# Autodesk Inventor assembly: SMALLER
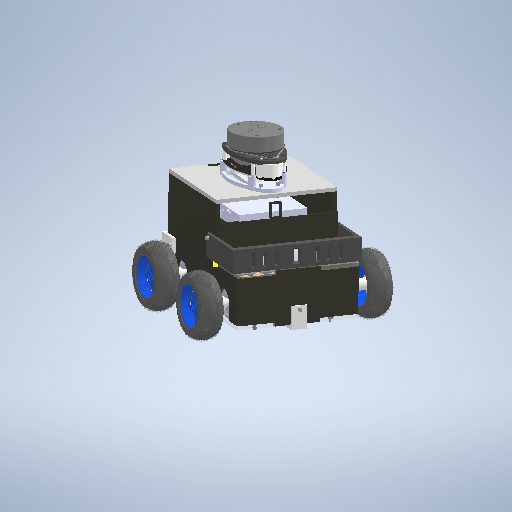
[picture p0: Inventor's stored thumbnail of the model, 512x512]
Saved by Autodesk Inventor 2025.3 (Build 293356030, 356C)
## iProperties
Created: 2026-06-30
Part Number: SMALLER
Document SubType Name: Assembly
Designer: user
Author: user
## Documents named in this file (14)
- C:\Users\user\Downloads\final_design\amy_robot_design.iam
- C:\Users\user\Downloads\final_design\motor_wheel\wheel_base.iam
- C:\Users\user\Downloads\final_design\chassis_boards\back.ipt
- C:\Users\user\Downloads\final_design\chassis_boards\Fastener.ipt
- C:\Users\user\Downloads\final_design\chassis_boards\side.ipt
- C:\Users\user\Downloads\final_design\chassis_boards\hood.ipt
- C:\Users\user\Downloads\final_design\chassis_boards\top.ipt
- C:\Users\user\Downloads\final_design\chassis_boards\front.ipt
- C:\Users\user\Downloads\final_design\chassis_boards\cover.ipt
- C:\Users\user\Downloads\final_design\chassis_boards\holder.ipt
- C:\Docs\shcool\dojo\CAD_stuff\Imports\assembled_lidar.iam
- C:\Docs\shcool\dojo\CAD_stuff\Design_3 - Copy\pi_internals\Complete_model.iam
- C:\Users\user\OneDrive\Documents\Inventor\Content Center Files\R2025\en-US\ISO 7040\DIEN EN ISO 7040 - M3.ipt
- C:\Users\user\OneDrive\Documents\Inventor\Content Center Files\R2025\en-US\ISO 4762(2)\ISO 4762 - M3 x 16ISO.ipt
## Components (48 placed, 13 different names)
1. wheel_base:1 [sub-assembly] — Mate:15, Mate:16, Mate:17, Mate:18, Mate:19, Insert:17
2. back:1 — Mate:5, Mate:6, Mate:7, Mate:8, Mate:9, Mate:12, Mate:14, Mate:15, Mate:21, Mate:23, Mate:24, Mate:25, Mate:26, Mate:27, Mate:28, Insert:25, Insert:29, Insert:30
3. side:1 — Mate:5, Mate:6, Mate:7, Mate:13, Mate:32, Mate:33, Insert:20, Insert:31
4. side:2 — Mate:8, Mate:9, Mate:16, Mate:20, Mate:22, Insert:28, Insert:34
5. Fastener:2 — Mate:20, Mate:21, Mate:22, Insert:7, Insert:8
6. Fastener:3 — Mate:12, Mate:13, Mate:14, Insert:9, Insert:10
7. Fastener:4 — Mate:17, Mate:18, Mate:19, Insert:3, Insert:4
8. hood:1 — Mate:23, Mate:24, Mate:30, Mate:31, Mate:47
9. top:1 — Mate:25, Mate:26, Mate:29, Insert:24, Mate:48, Insert:39, Insert:40, Insert:41, Insert:42
10. Fastener:5 — Mate:27, Mate:28, Mate:29, Insert:5, Insert:6
11. front:1 — Mate:30, Mate:31, Mate:34, Mate:35, Mate:36
12. cover:1 — Mate:32, Mate:33, Mate:42, Mate:43
13. Fastener:6 — Mate:34, Mate:35, Mate:36, Insert:1, Insert:2, Insert:18
14. holder:1 — Mate:47, Insert:32, Insert:33
15. Complete_model:1 [sub-assembly] — Mate:42, Mate:43
16. DIN EN ISO 7040 M3:1 — Insert:18
17. ISO 4762 M3 x 16:2 — Insert:4
18. ISO 4762 M3 x 16:3 — Insert:3
19. ISO 4762 M3 x 16:4 — Insert:1, Insert:27
20. ISO 4762 M3 x 16:5 — Insert:2
21. DIN EN ISO 7040 M3:2 — Insert:17
22. DIN EN ISO 7040 M3:3 — Insert:31
23. DIN EN ISO 7040 M3:4
24. DIN EN ISO 7040 M3:5 — Insert:20
25. ISO 4762 M3 x 16:6 — Insert:10
26. ISO 4762 M3 x 16:7 — Insert:9
27. ISO 4762 M3 x 16:8 — Insert:5
28. ISO 4762 M3 x 16:9 — Insert:8
29. ISO 4762 M3 x 16:10 — Insert:7
30. ISO 4762 M3 x 16:11 — Insert:6
31. DIN EN ISO 7040 M3:6 — Insert:27
32. DIN EN ISO 7040 M3:11 — Insert:24
33. DIN EN ISO 7040 M3:12 — Insert:25
34. DIN EN ISO 7040 M3:13 — Insert:28
35. DIN EN ISO 7040 M3:14 — Insert:29
36. DIN EN ISO 7040 M3:15 — Insert:30
37. DIN EN ISO 7040 M3:17 — Insert:34
38. ISO 4762 M3 x 16:16 — Insert:32
39. ISO 4762 M3 x 16:17 — Insert:33
40. assembled_lidar:1 [sub-assembly] — Mate:48, Insert:35, Insert:36, Insert:37, Insert:38
41. ISO 4762 M3 x 16:18 — Insert:38
42. DIN EN ISO 7040 M3:18 — Insert:39
43. ISO 4762 M3 x 16:19 — Insert:36
44. ISO 4762 M3 x 16:20 — Insert:35
45. ISO 4762 M3 x 16:21 — Insert:37
46. DIN EN ISO 7040 M3:19 — Insert:42
47. DIN EN ISO 7040 M3:20 — Insert:41
48. DIN EN ISO 7040 M3:21 — Insert:40
## Relationships (65: Mate 34, Insert 31)
- Mate:5: back:1 ↔ side:1
- Mate:6: back:1 ↔ side:1
- Mate:7: back:1 ↔ side:1
- Mate:8: back:1 ↔ side:2
- Mate:9: back:1 ↔ side:2
- Mate:12: back:1 ↔ Fastener:3
- Mate:13: side:1 ↔ Fastener:3
- Mate:14: back:1 ↔ Fastener:3
- Mate:15: wheel_base:1 ↔ back:1
- Mate:16: wheel_base:1 ↔ side:2
- Mate:17: wheel_base:1 ↔ Fastener:4
- Mate:18: wheel_base:1 ↔ Fastener:4
- Mate:19: wheel_base:1 ↔ Fastener:4
- Mate:20: side:2 ↔ Fastener:2
- Mate:21: back:1 ↔ Fastener:2
- Mate:22: side:2 ↔ Fastener:2
- Mate:23: back:1 ↔ hood:1
- Mate:24: back:1 ↔ hood:1
- Mate:25: back:1 ↔ top:1
- Mate:26: back:1 ↔ top:1
- Mate:27: back:1 ↔ Fastener:5
- Mate:28: back:1 ↔ Fastener:5
- Mate:29: top:1 ↔ Fastener:5
- Mate:30: hood:1 ↔ front:1
- Mate:31: hood:1 ↔ front:1
- Mate:32: side:1 ↔ cover:1
- Mate:33: side:1 ↔ cover:1
- Mate:34: front:1 ↔ Fastener:6
- Mate:35: front:1 ↔ Fastener:6
- Mate:36: front:1 ↔ Fastener:6
- Mate:42: cover:1 ↔ Complete_model:1
- Mate:43: cover:1 ↔ Complete_model:1
- Insert:1: Fastener:6 ↔ ISO 4762 M3 x 16:4
- Insert:2: Fastener:6 ↔ ISO 4762 M3 x 16:5
- Insert:3: Fastener:4 ↔ ISO 4762 M3 x 16:3
- Insert:4: Fastener:4 ↔ ISO 4762 M3 x 16:2
- Insert:5: Fastener:5 ↔ ISO 4762 M3 x 16:8
- Insert:6: Fastener:5 ↔ ISO 4762 M3 x 16:11
- Insert:7: Fastener:2 ↔ ISO 4762 M3 x 16:10
- Insert:8: Fastener:2 ↔ ISO 4762 M3 x 16:9
- Insert:9: Fastener:3 ↔ ISO 4762 M3 x 16:7
- Insert:10: Fastener:3 ↔ ISO 4762 M3 x 16:6
- Insert:17: wheel_base:1 ↔ DIN EN ISO 7040 M3:2
- Insert:18: Fastener:6 ↔ DIN EN ISO 7040 M3:1
- Insert:20: side:1 ↔ DIN EN ISO 7040 M3:5
- Insert:24: top:1 ↔ DIN EN ISO 7040 M3:11
- Insert:25: back:1 ↔ DIN EN ISO 7040 M3:12
- Insert:27: ISO 4762 M3 x 16:4 ↔ DIN EN ISO 7040 M3:6
- Insert:28: side:2 ↔ DIN EN ISO 7040 M3:13
- Insert:29: back:1 ↔ DIN EN ISO 7040 M3:14
- Insert:30: back:1 ↔ DIN EN ISO 7040 M3:15
- Insert:31: side:1 ↔ DIN EN ISO 7040 M3:3
- Mate:47: hood:1 ↔ holder:1
- Insert:32: holder:1 ↔ ISO 4762 M3 x 16:16
- Insert:33: holder:1 ↔ ISO 4762 M3 x 16:17
- Insert:34: side:2 ↔ DIN EN ISO 7040 M3:17
- Mate:48: top:1 ↔ assembled_lidar:1
- Insert:35: assembled_lidar:1 ↔ ISO 4762 M3 x 16:20
- Insert:36: assembled_lidar:1 ↔ ISO 4762 M3 x 16:19
- Insert:37: assembled_lidar:1 ↔ ISO 4762 M3 x 16:21
- Insert:38: assembled_lidar:1 ↔ ISO 4762 M3 x 16:18
- Insert:39: top:1 ↔ DIN EN ISO 7040 M3:18
- Insert:40: top:1 ↔ DIN EN ISO 7040 M3:21
- Insert:41: top:1 ↔ DIN EN ISO 7040 M3:20
- Insert:42: top:1 ↔ DIN EN ISO 7040 M3:19
